# Autodesk Inventor assembly: Assembly_Cube_openISM_Anybeam
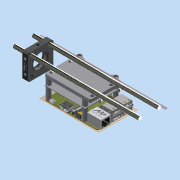
[picture p0: Inventor's stored thumbnail of the model, 180x180]
Saved by Autodesk Inventor 2019.4 (Build 234330000, 330)
## iProperties
Created: 2020-12-16
Part Number: Assembly_Cube_openISM_Anybeam
Document SubType Name: Assembly
Designer: diederichbenedict
Author: diederichbenedict
## Documents named in this file (7)
- C:\Users\diederichbenedict\Dropbox\Dokumente\Promotion\PROJECTS\UC2\02_CAD\INVENTOR\uc2_v3\Assembly_Cube_openISM_Anybeam.iam
- C:\Users\diederichbenedict\Dropbox\Dokumente\Promotion\PROJECTS\UC2\02_CAD\INVENTOR\uc2_v3\00_Anybeam_Nebra_HAT.ipt
- C:\Users\diederichbenedict\Dropbox\Dokumente\Promotion\PROJECTS\UC2\02_CAD\INVENTOR\uc2_v3\00_Raspi.ipt
- C:\Users\diederichbenedict\Dropbox\Dokumente\Promotion\PROJECTS\UC2\02_CAD\INVENTOR\uc2_v3\20_Cube_insert_openISM_AnyBeamMount.ipt
- C:\Users\diederichbenedict\Dropbox\Dokumente\Promotion\PROJECTS\UC2\02_CAD\INVENTOR\uc2_v3\00_BallMagnets_5mm_single.ipt
- C:\Users\diederichbenedict\Dropbox\Dokumente\Promotion\PROJECTS\UC2\02_CAD\INVENTOR\uc2_v3\00_Thorlabs_Cage_CP33_M.ipt
- C:\Users\diederichbenedict\Dropbox\Dokumente\Promotion\PROJECTS\UC2\02_CAD\INVENTOR\uc2_v3\00_Thorlabs_Rod_200mm.ipt
## Components (14 placed, 6 different names)
1. 20_Cube_insert_openISM_AnyBeamMount:1 — Flush:1
2. 00_Thorlabs_Cage_CP33_M:1 — Insert:1, Angle:3
3. 00_Thorlabs_Rod_200mm:2
4. 00_Thorlabs_Rod_200mm:1
5. 00_Anybeam_Nebra_HAT:1 — Insert:1, Angle:3, Flush:1, Insert:2, Insert:3
6. 00_Raspi:1 — Insert:2, Insert:3
7. 00_BallMagnets_5mm_single:2
8. 00_BallMagnets_5mm_single:1
9. 00_BallMagnets_5mm_single:3
10. 00_BallMagnets_5mm_single:4
11. 00_BallMagnets_5mm_single:5
12. 00_BallMagnets_5mm_single:6
13. 00_BallMagnets_5mm_single:7
14. 00_BallMagnets_5mm_single:8
## Component patterns: (2 elements), (2 elements, first: 00_BallMagnets_5mm_single:2 + 00_BallMagnets_5mm_single:1), Component Pattern 1:2 (2 elements)
## Relationships (16: Tangent 6, Mate 4, Insert 3, Angle 2, Flush 1)
- [Mate]: 20_Cube_insert_openISM_AnyBeamMount:1 ↔ 00_BallMagnets_5mm_single:1
- [Tangent]: 20_Cube_insert_openISM_AnyBeamMount:1 ↔ 00_BallMagnets_5mm_single:1
- [Mate]: 20_Cube_insert_openISM_AnyBeamMount:1 ↔ 00_BallMagnets_5mm_single:2
- [Tangent]: 20_Cube_insert_openISM_AnyBeamMount:1 ↔ 00_BallMagnets_5mm_single:2
- [Angle] (180 deg): 20_Cube_insert_openISM_AnyBeamMount:1 ↔ 00_Thorlabs_Cage_CP33_M:1
- Insert:1 (40 mm): 00_Thorlabs_Cage_CP33_M:1 ↔ 00_Anybeam_Nebra_HAT:1
- Angle:3 (180 deg): 00_Thorlabs_Cage_CP33_M:1 ↔ 00_Anybeam_Nebra_HAT:1
- [Mate]: 00_Thorlabs_Cage_CP33_M:1 ↔ 00_Thorlabs_Rod_200mm:2
- [Mate]: 00_Thorlabs_Cage_CP33_M:1 ↔ 00_Thorlabs_Rod_200mm:1
- [Tangent]: 00_Thorlabs_Rod_200mm:2 ↔ 00_BallMagnets_5mm_single:3
- [Tangent]: 00_Thorlabs_Rod_200mm:2 ↔ 00_BallMagnets_5mm_single:4
- [Tangent]: 00_Thorlabs_Rod_200mm:1 ↔ 00_BallMagnets_5mm_single:6
- [Tangent]: 00_Thorlabs_Rod_200mm:2 ↔ 00_BallMagnets_5mm_single:7
- Flush:1: 20_Cube_insert_openISM_AnyBeamMount:1 ↔ 00_Anybeam_Nebra_HAT:1
- Insert:2: 00_Anybeam_Nebra_HAT:1 ↔ 00_Raspi:1
- Insert:3: 00_Anybeam_Nebra_HAT:1 ↔ 00_Raspi:1
## Named parameters: d28_d30 = 0 mm, d29_d13 = 0 mm, d30_d14 = 0 mm
